# Autodesk Inventor assembly: 4Pin_Set
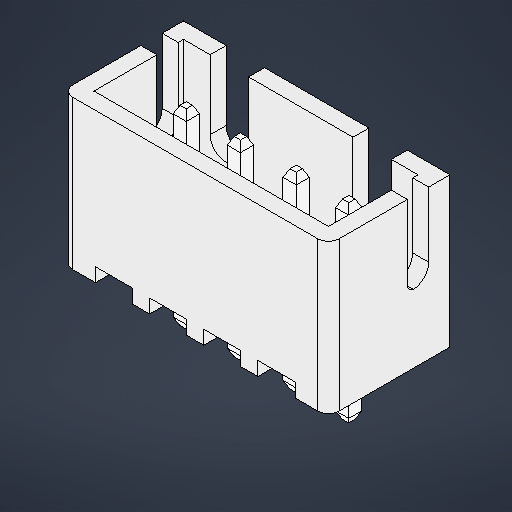
[picture p0: Inventor's stored thumbnail of the model, 512x512]
Saved by Autodesk Inventor 2026 (Build 300175000, 175)
## iProperties
Created: 2025-04-18
Part Number: 4Pin_Set
Document SubType Name: Assembly
Designer: ct_vi
Author: ct_vi
## Documents named in this file (3)
- C:\Users\ct_vi\Documents\Capstone_Research_3D_Files\4Pin_Set.iam
- C:\Users\ct_vi\Documents\Capstone_Research_3D_Files\4pin_head.ipt
- C:\Users\ct_vi\Documents\Capstone_Research_3D_Files\Pin_Header.ipt
## Components (5 placed, 2 different names)
1. 4pin_head:1 — Mate:1, Flush:1, Mate:2, Mate:3, Flush:2, Mate:4, Mate:5, Flush:3, Mate:6, Mate:7, Flush:4
2. Pin_Header:1 — Mate:1, Flush:1, Mate:2
3. Pin_Header:3 — Mate:3, Flush:2
4. Pin_Header:4 — Mate:4, Mate:5, Flush:3
5. Pin_Header:5 — Mate:6, Mate:7, Flush:4
## Relationships (11: Mate 7, Flush 4)
- Mate:1: 4pin_head:1 ↔ Pin_Header:1
- Flush:1 (-3 mm): 4pin_head:1 ↔ Pin_Header:1
- Mate:2: 4pin_head:1 ↔ Pin_Header:1
- Mate:3: 4pin_head:1 ↔ Pin_Header:3
- Flush:2 (-3 mm): 4pin_head:1 ↔ Pin_Header:3
- Mate:4: 4pin_head:1 ↔ Pin_Header:4
- Mate:5: 4pin_head:1 ↔ Pin_Header:4
- Flush:3 (-3 mm): 4pin_head:1 ↔ Pin_Header:4
- Mate:6: 4pin_head:1 ↔ Pin_Header:5
- Mate:7: 4pin_head:1 ↔ Pin_Header:5
- Flush:4 (-3 mm): 4pin_head:1 ↔ Pin_Header:5
